# Autodesk Inventor assembly: KND-2600 DrainSystemBottom 01
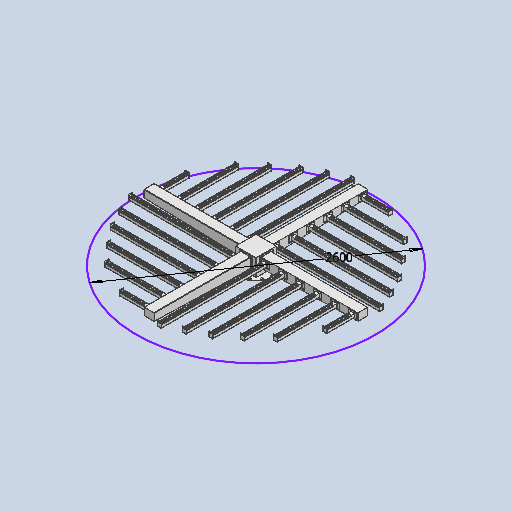
[picture p0: Inventor's stored thumbnail of the model, 512x512]
Saved by Autodesk Inventor 2026.2 (Build 302298000, 298)
## iProperties
Created: 2026-05-12
Part Number: KND-2600 DrainSystemBottom 01
Document SubType Name: Assembly
Designer: admin
Stock Number: ДРС Ф2600
Author: admin
## Documents named in this file (4)
- C:\Users\admin\Documents\Inventor\KND-DistribSystem\DRS_D1200\KND-2600 DrainSystemBottom 01.iam
- C:\Users\admin\Documents\Inventor\KND-DistribSystem\DRS_D1200\KND-1401 DrSysB DIMentions 01.ipt
- C:\Users\admin\Documents\Inventor\KND-DistribSystem\DRS_D1200\KND-1000 Center 01.iam
- C:\Users\admin\Documents\Inventor\KND-DistribSystem\DRS_D1200\KND-2000 Collector 01.iam
## Components (7 placed, 4 different names)
1. PRS 1401 DrSysB DIMentions_D1200:1
2. KND-1401 DrSysB DIMentions 01:2
3. KND-1000 Center 01:1 [sub-assembly] — Mate:1, Mate:2, Mate:3, Mate:4, Mate:5, Mate:6, Mate:7, Mate:8, Mate:9, Mate:10, Mate:11, Mate:12
4. KND-2000 Collector 01:1 [sub-assembly] — Mate:1, Mate:2, Mate:3
5. KND-2000 Collector 01:2 [sub-assembly] — Mate:4, Mate:5, Mate:6
6. KND-2000 Collector 01:3 [sub-assembly] — Mate:7, Mate:8, Mate:9
7. KND-2000 Collector 01:4 [sub-assembly] — Mate:10, Mate:11, Mate:12
## Relationships (12: Mate 12)
- Mate:1: KND-1000 Center 01:1 ↔ KND-2000 Collector 01:1
- Mate:2 (0.2 mm): KND-1000 Center 01:1 ↔ KND-2000 Collector 01:1
- Mate:3 (0.25 mm): KND-1000 Center 01:1 ↔ KND-2000 Collector 01:1
- Mate:4: KND-1000 Center 01:1 ↔ KND-2000 Collector 01:2
- Mate:5 (0.2 mm): KND-1000 Center 01:1 ↔ KND-2000 Collector 01:2
- Mate:6 (0.25 mm): KND-1000 Center 01:1 ↔ KND-2000 Collector 01:2
- Mate:7: KND-1000 Center 01:1 ↔ KND-2000 Collector 01:3
- Mate:8 (0.2 mm): KND-1000 Center 01:1 ↔ KND-2000 Collector 01:3
- Mate:9 (0.3 mm): KND-1000 Center 01:1 ↔ KND-2000 Collector 01:3
- Mate:10: KND-1000 Center 01:1 ↔ KND-2000 Collector 01:4
- Mate:11 (0.3 mm): KND-1000 Center 01:1 ↔ KND-2000 Collector 01:4
- Mate:12 (0.3 mm): KND-1000 Center 01:1 ↔ KND-2000 Collector 01:4
